# Autodesk Inventor assembly: LAUNCHPAD ASSEMBLY
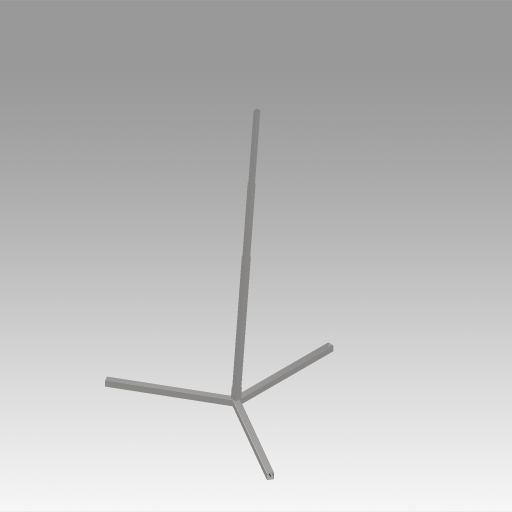
[picture p0: Inventor's stored thumbnail of the model, 512x512]
Saved by Autodesk Inventor 2023 (Build 270158000, 158)
## iProperties
_SolveAssemblyDoc: Frame Generator Solve Assembly
_Version: 25.0.0
Created: 2025-04-04
Part Number: LAUNCHPAD ASSEMBLY
Document SubType Name: Assembly
Designer: NELLY NDUNG'U
Author: NELLY NDUNG'U
## Documents named in this file (10)
- N:\NAKUJA\CAD FILES\AIRFRAME\LP001\LAUNCHPAD ASSEMBLY.iam
- N:\NAKUJA\CAD FILES\AIRFRAME\LP001\BASE.ipt
- N:\NAKUJA\CAD FILES\AIRFRAME\LP001\LAUNCHPAD ASSEMBLY\Frame\Frame 1743750012638.iam
- N:\NAKUJA\CAD FILES\AIRFRAME\LP001\LP01.iam
- N:\NAKUJA\CAD FILES\AIRFRAME\LP001\LP02.iam
- N:\NAKUJA\CAD FILES\AIRFRAME\LP001\LP02_2.iam
- C:\Users\User\Documents\Inventor\Content Center Files\R2023\en-US\ANSI B18.2.3.5M\ANSI B18.2.3.5M - M10 x 1.5 x 100.ipt
- C:\Users\User\Documents\Inventor\Content Center Files\R2023\en-US\ANSI B 18.2.4.1 M(1)\ANSI B 18.2.4.1 M - M10 x 1.5Style 1.ipt
- C:\Users\User\Documents\Inventor\Content Center Files\R2023\en-US\ANSI B18.2.3.5M\ANSI B18.2.3.5M - M10 x 1.5 x 90.ipt
- C:\Users\User\Documents\Inventor\Content Center Files\R2023\en-US\ANSI B18.2.3.5M\ANSI B18.2.3.5M - M10 x 1.5 x 80.ipt
## Components (19 placed, 9 different names)
1. BASE:1
2. Frame 1743750012638:1 [sub-assembly] — Mate:10, Mate:11, Mate:12, Insert:1, Insert:2, Insert:3, Insert:4, Insert:5
3. LP01:1 [sub-assembly] — Mate:4, Mate:5, Mate:6, Mate:10, Mate:11, Mate:12, Insert:6, Insert:7, Insert:8, Insert:9
4. LP02:1 [sub-assembly] — Mate:4, Mate:5, Mate:6, Mate:7, Mate:8, Mate:9, Insert:10, Insert:11, Insert:12, Insert:13
5. LP02_2:1 [sub-assembly] — Mate:7, Mate:8, Mate:9
6. Hex Bolt - Metric M10 x 1.5 x 100:1 — Insert:2
7. Hex Bolt - Metric M10 x 1.5 x 100:2 — Insert:1
8. Hex Bolt - Metric M10 x 1.5 x 100:3 — Insert:3
9. Hex Nut Metric M10 x 1.5:1 — Insert:5
10. Hex Nut Metric M10 x 1.5:2 — Insert:4
11. Hex Nut Metric M10 x 1.5:3
12. Hex Bolt - Metric M10 x 1.5 x 90:1 — Insert:6
13. Hex Bolt - Metric M10 x 1.5 x 90:2 — Insert:7
14. Hex Nut Metric M10 x 1.5:4 — Insert:8
15. Hex Nut Metric M10 x 1.5:5 — Insert:9
16. Hex Bolt - Metric M10 x 1.5 x 80:1 — Insert:10
17. Hex Bolt - Metric M10 x 1.5 x 80:2 — Insert:11
18. Hex Nut Metric M10 x 1.5:6 — Insert:12
19. Hex Nut Metric M10 x 1.5:7 — Insert:13
## Relationships (22: Insert 13, Mate 9)
- Mate:4 (2 mm): LP01:1 ↔ LP02:1
- Mate:5 (2 mm): LP01:1 ↔ LP02:1
- Mate:6 (-125 mm): LP01:1 ↔ LP02:1
- Mate:7 (2 mm): LP02:1 ↔ LP02_2:1
- Mate:8 (2 mm): LP02:1 ↔ LP02_2:1
- Mate:9 (-125 mm): LP02:1 ↔ LP02_2:1
- Mate:10 (2 mm): Frame 1743750012638:1 ↔ LP01:1
- Mate:11 (2 mm): Frame 1743750012638:1 ↔ LP01:1
- Mate:12 (-162 mm): Frame 1743750012638:1 ↔ LP01:1
- Insert:1: Frame 1743750012638:1 ↔ Hex Bolt - Metric M10 x 1.5 x 100:2
- Insert:2: Frame 1743750012638:1 ↔ Hex Bolt - Metric M10 x 1.5 x 100:1
- Insert:3: Frame 1743750012638:1 ↔ Hex Bolt - Metric M10 x 1.5 x 100:3
- Insert:4: Frame 1743750012638:1 ↔ Hex Nut Metric M10 x 1.5:2
- Insert:5: Frame 1743750012638:1 ↔ Hex Nut Metric M10 x 1.5:1
- Insert:6: LP01:1 ↔ Hex Bolt - Metric M10 x 1.5 x 90:1
- Insert:7: LP01:1 ↔ Hex Bolt - Metric M10 x 1.5 x 90:2
- Insert:8: LP01:1 ↔ Hex Nut Metric M10 x 1.5:4
- Insert:9: LP01:1 ↔ Hex Nut Metric M10 x 1.5:5
- Insert:10: LP02:1 ↔ Hex Bolt - Metric M10 x 1.5 x 80:1
- Insert:11: LP02:1 ↔ Hex Bolt - Metric M10 x 1.5 x 80:2
- Insert:12: LP02:1 ↔ Hex Nut Metric M10 x 1.5:6
- Insert:13: LP02:1 ↔ Hex Nut Metric M10 x 1.5:7
